# Autodesk Inventor assembly: main_idea
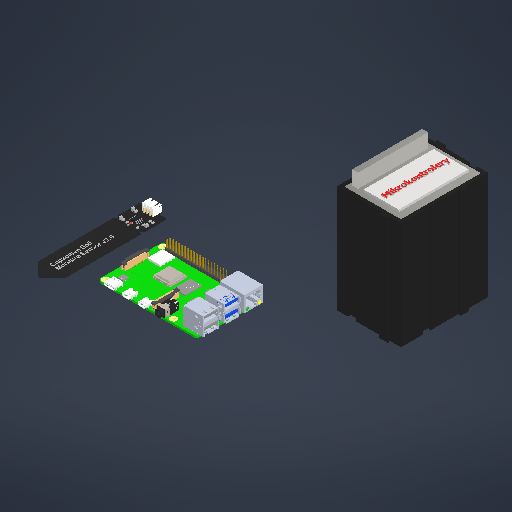
[picture p0: Inventor's stored thumbnail of the model, 512x512]
Saved by Autodesk Inventor 2027 (Build 310192060, 192F)
## iProperties
Created: 2026-06-08
Part Number: main_idea
Document SubType Name: Assembly
Designer: User
Author: User
## Documents named in this file (6)
- C:\Users\Duszy\Desktop\Modular_shelf\main_idea.iam
- C:\Users\Duszy\Desktop\Modular_shelf\Parts\box.ipt
- C:\Users\Duszy\Desktop\Modular_shelf\Parts\shelf.ipt
- C:\Users\Duszy\Desktop\Modular_shelf\Parts\example of items\Moisture Sensor\Moisture Sensor.ipt
- C:\Users\Duszy\Desktop\Shelf\example of items\NUCLEO-F411RE\NUCLEO-F411RE.ipt
- C:\Users\Duszy\Desktop\Modular_shelf\Parts\example of items\Raspberry Pi 4 Model B\Raspberry Pi 4 Model B.ipt
## Components (5 placed, 5 different names)
1. box:1 — Walcowe:1
2. shelf:1 — Walcowe:1
3. Moisture Sensor:1
4. NUCLEO-F411RE:1
5. Raspberry Pi 4 Model B:1
## Relationships (1: CylindricalJoint 1)
- Walcowe:1 [CylindricalJoint]: box:1 ↔ shelf:1
